# Autodesk Inventor assembly: ReleaseAssembly
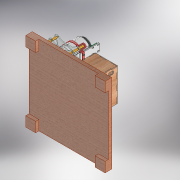
[picture p0: Inventor's stored thumbnail of the model, 180x180]
Saved by Autodesk Inventor 2018.2 (Build 222227000, 227)
## iProperties
Created: 2018-03-27
Part Number: ReleaseAssembly
Document SubType Name: Assembly
Designer: mansu
Author: mansu
## Documents named in this file (13)
- C:\Users\Moochster\OneDrive\Documents\2018 UBC\ELEC 391\Controller\cad\release\ReleaseAssembly.iam
- C:\Users\Moochster\OneDrive\Documents\2018 UBC\ELEC 391\Controller\cad\release\PitchAssembly.iam
- C:\Users\Moochster\OneDrive\Documents\2018 UBC\ELEC 391\Controller\cad\release\YawAssembly.iam
- C:\Users\Moochster\OneDrive\Documents\2018 UBC\ELEC 391\Controller\cad\release\WoodBase.ipt
- C:\Users\Moochster\OneDrive\Documents\2018 UBC\ELEC 391\Controller\cad\release\pcb.iam
- C:\Users\Moochster\OneDrive\Documents\2018 UBC\ELEC 391\Controller\cad\release\Fasteners\StandoffM4x5B.ipt
- C:\Users\Moochster\OneDrive\Documents\2018 UBC\ELEC 391\Controller\cad\release\ControlBoxTop.ipt
- C:\Users\Moochster\OneDrive\Documents\2018 UBC\ELEC 391\Controller\cad\release\ControlBoxFace.ipt
- C:\Users\Moochster\OneDrive\Documents\2018 UBC\ELEC 391\Controller\cad\release\40x40x10 DC Fan.ipt
- C:\Users\Moochster\OneDrive\Documents\2018 UBC\ELEC 391\Controller\cad\release\ControlBoxFlatFace.ipt
- C:\Users\Moochster\OneDrive\Documents\2018 UBC\ELEC 391\Controller\cad\release\ControlBoxSide.ipt
- C:\Users\Moochster\OneDrive\Documents\2018 UBC\ELEC 391\Controller\cad\release\ControlBoxSidePower.ipt
- C:\Users\Moochster\OneDrive\Documents\2018 UBC\ELEC 391\Controller\cad\release\ShaftBushing.ipt
## Components (16 placed, 12 different names)
1. PitchAssembly:1 [sub-assembly] — Flush:1, Mate:24, Mate:25
2. YawAssembly:1 [sub-assembly] — Mate:1, Flush:1, Mate:26
3. WoodBase:1 — Mate:3, Mate:23, Angle:1, Mate:26
4. pcb:1 [sub-assembly] — Insert:1, Insert:2, Insert:3, Insert:4
5. StandoffM4x5B:1 — Insert:3, Mate:3
6. StandoffM4x5B:2 — Insert:1
7. StandoffM4x5B:3 — Insert:4
8. StandoffM4x5B:4 — Insert:2
9. ControlBoxTop:1 — Flush:5, Flush:6, Flush:8, Flush:9
10. ControlBoxFlatFace:1 — Flush:5, Mate:17, Mate:18, Mate:19, Mate:20, Flush:8, Mate:23, Angle:1
11. ControlBoxFace:2 — Flush:6, Mate:12, Mate:13, Mate:14, Mate:15, Mate:16, Mate:21, Mate:22
12. 40x40x10 DC Fan:1 — Mate:12, Flush:7, Mate:14, Mate:15
13. 40x40x10 DC Fan:2 — Mate:13, Flush:7, Mate:16
14. ControlBoxSidePower:1 — Mate:17, Mate:18, Mate:21, Mate:22, Flush:9
15. ControlBoxSide:2 — Mate:19, Mate:20
16. ShaftBushing:1 — Mate:24, Mate:25
## Relationships (28: Mate 17, Flush 6, Insert 4, Angle 1)
- Mate:1: YawAssembly:1
- Flush:1: PitchAssembly:1 ↔ YawAssembly:1
- Insert:1: pcb:1 ↔ StandoffM4x5B:2
- Insert:2: pcb:1 ↔ StandoffM4x5B:4
- Insert:3: pcb:1 ↔ StandoffM4x5B:1
- Insert:4: pcb:1 ↔ StandoffM4x5B:3
- Mate:3: WoodBase:1 ↔ StandoffM4x5B:1
- Flush:5: ControlBoxTop:1 ↔ ControlBoxFlatFace:1
- Flush:6: ControlBoxTop:1 ↔ ControlBoxFace:2
- Mate:12: ControlBoxFace:2 ↔ 40x40x10 DC Fan:1
- Mate:13: ControlBoxFace:2 ↔ 40x40x10 DC Fan:2
- Flush:7: 40x40x10 DC Fan:1 ↔ 40x40x10 DC Fan:2
- Mate:14: ControlBoxFace:2 ↔ 40x40x10 DC Fan:1
- Mate:15: ControlBoxFace:2 ↔ 40x40x10 DC Fan:1
- Mate:16: ControlBoxFace:2 ↔ 40x40x10 DC Fan:2
- Mate:17: ControlBoxFlatFace:1 ↔ ControlBoxSidePower:1
- Mate:18: ControlBoxFlatFace:1 ↔ ControlBoxSidePower:1
- Mate:19: ControlBoxFlatFace:1 ↔ ControlBoxSide:2
- Mate:20: ControlBoxFlatFace:1 ↔ ControlBoxSide:2
- Mate:21: ControlBoxFace:2 ↔ ControlBoxSidePower:1
- Mate:22: ControlBoxFace:2 ↔ ControlBoxSidePower:1
- Flush:8: ControlBoxTop:1 ↔ ControlBoxFlatFace:1
- Flush:9: ControlBoxTop:1 ↔ ControlBoxSidePower:1
- Mate:23: WoodBase:1 ↔ ControlBoxFlatFace:1
- Angle:1 (0 deg): WoodBase:1 ↔ ControlBoxFlatFace:1
- Mate:24: PitchAssembly:1 ↔ ShaftBushing:1
- Mate:25 (0.1 mm): PitchAssembly:1 ↔ ShaftBushing:1
- Mate:26: YawAssembly:1 ↔ WoodBase:1
